# Autodesk Inventor assembly: (Unsaved)
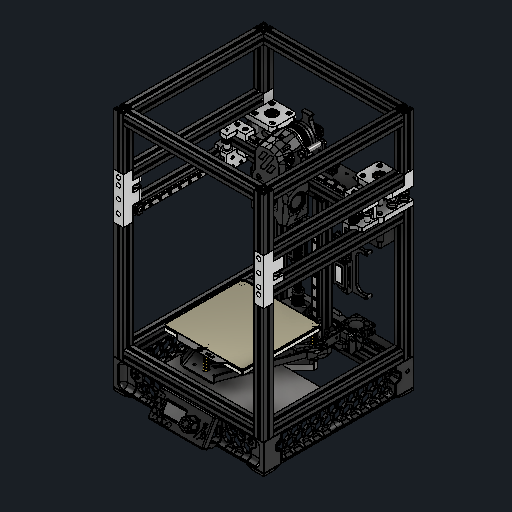
[picture p0: Inventor's stored thumbnail of the model, 512x512]
Saved by Autodesk Inventor 2026.2 (Build 302298000, 298)
## iProperties
Created: 2025-05-09
Part Number: (Unsaved)
Document SubType Name: Assembly
Designer: AdminForWorker
Title: Voron 0 v2
Author: AdminForWorker
## Documents named in this file (19)
- C:\Users\JoshuaEah\Documents\GitHub\Voron-0\CAD\Voron 0.iam
- C:\Users\JoshuaEah\Documents\GitHub\Voron-0\CAD\Frame\Frame.iam
- C:\Users\JoshuaEah\Documents\GitHub\Voron-0\CAD\Skirt\Skirts.iam
- C:\Users\JoshuaEah\Documents\GitHub\Voron-0\CAD\Hardware\Electronics\Electronics.iam
- C:\Users\JoshuaEah\Documents\GitHub\Voron-0\CAD\Extras\Filament Spool.iam
- C:\Users\JoshuaEah\Documents\GitHub\Voron-0\CAD\Z Axis\Bed Assembly.iam
- C:\Users\JoshuaEah\Documents\GitHub\Voron-0\CAD\Z Axis\Z Motor Assembly.iam
- C:\Users\JoshuaEah\Documents\GitHub\Voron-0\CAD\Z Axis\Z Extrusion Right.iam
- Z Extrusion Right.iam
- C:\Users\JoshuaEah\Documents\GitHub\Voron-0\CAD\Z Axis\Z Extrusion Left.iam
- C:\Users\JoshuaEah\Documents\GitHub\Voron-0\CAD\Hardware\Linear Rail\Parts\MGN7H Carriage.ipt
- C:\Users\JoshuaEah\Documents\GitHub\Voron-0\CAD\Belts\Belts.iam
- C:\Users\JoshuaEah\Documents\GitHub\Voron-0\CAD\X Axis\X Axis.iam
- C:\Users\JoshuaEah\Documents\GitHub\Voron-0\CAD\Toolhead\Mini Stealthburner.iam
- C:\Users\JoshuaEah\Documents\GitHub\Voron-0\CAD\Enclosure\Enclosure.iam
- C:\Users\JoshuaEah\Documents\GitHub\Voron-0\CAD\AB Drives\A_Drive.iam
- C:\Users\JoshuaEah\Documents\GitHub\Voron-0\CAD\AB Drives\B_Drive.iam
- C:\Users\JoshuaEah\Documents\GitHub\Voron-0\CAD\Idlers\A Idler Assembly (Alternate).iam
- C:\Users\JoshuaEah\Documents\GitHub\Voron-0\CAD\Idlers\B Idler Assembly (Alternate).iam
## Components (21 placed, 21 different names)
1. Frame:1 [sub-assembly] — Flush:3, Angle:1, Mate:4, Cylindrical:5, Insert:7, Insert:8, Mate:22, Mate:23, Angle:3, Cylindrical:13, Angle:4, Insert:17, Insert:18, Insert:19, Insert:20
2. Belts:1 [sub-assembly] — Mate:24
3. A_Drive:1 [sub-assembly] — Insert:7, Mate:23
4. B_Drive:1 [sub-assembly] — Insert:8, Mate:22
5. X Axis:1 [sub-assembly] — Insert:13, Insert:14, Cylindrical:12, Angle:2, Mate:24
6. MGN7H X Carriage:1 — Cylindrical:12, Insert:15, Insert:16, Angle:2
7. Mini Stealthburner:1 [sub-assembly] — Insert:15, Insert:16
8. MGN7H Y Left Carriage:1 — Cylindrical:5, Insert:13, Angle:3
9. MGN7H Y Right Carriage:1 — Insert:14, Cylindrical:13, Angle:4
10. Bed Assembly:1 [sub-assembly] — Mate:1, Insert:1, Insert:2, Insert:3, Insert:4
11. Z Motor Assembly:1 [sub-assembly] — Mate:1, Flush:3, Angle:1
12. Z Extrusion Right:1 [sub-assembly] — Cylindrical:15, Angle:6
13. Z Extrusion Left:1 [sub-assembly] — Mate:4, Cylindrical:14, Angle:5
14. MGN7H Z Left Carriage:1 — Insert:2, Insert:3, Cylindrical:14, Angle:5
15. MGN7H Z Right Carriage:1 — Insert:1, Insert:4, Cylindrical:15, Angle:6
16. Skirts:1 [sub-assembly]
17. Enclosure:1 [sub-assembly]
18. Electronics:1 [sub-assembly]
19. Filament Spool:1 [sub-assembly]
20. A Idler Assembly (Alternate):1 [sub-assembly] — Insert:17, Insert:18
21. B Idler Assembly (Alternate):1 [sub-assembly] — Insert:19, Insert:20
## Relationships (53: Mate 18, Insert 14, Flush 10, Angle 6, CylindricalJoint 5)
- Mate:1: Bed Assembly:1 ↔ Z Motor Assembly:1
- [Mate]: Frame:1 ↔ Z Extrusion Right:1
- [Mate]: Frame:1 ↔ Z Extrusion Left:1
- [Flush]: Frame:1 ↔ Z Extrusion Right:1
- [Flush]: Frame:1 ↔ Z Extrusion Left:1
- Insert:1: Bed Assembly:1 ↔ MGN7H Z Right Carriage:1
- Insert:2: Bed Assembly:1 ↔ MGN7H Z Left Carriage:1
- Insert:3: Bed Assembly:1 ↔ MGN7H Z Left Carriage:1
- Insert:4: Bed Assembly:1 ↔ MGN7H Z Right Carriage:1
- Flush:3: Frame:1 ↔ Z Motor Assembly:1
- Angle:1 (0 deg): Frame:1 ↔ Z Motor Assembly:1
- Mate:4 (58 mm): Frame:1 ↔ Z Extrusion Left:1
- [Flush]: Bed Assembly:1 ↔ Z Extrusion Right:1
- Cylindrical:5: Frame:1 ↔ MGN7H Y Left Carriage:1
- [Mate]: Frame:1 ↔ Enclosure:1
- [Flush]: Frame:1 ↔ Enclosure:1
- [Flush]: Frame:1 ↔ Enclosure:1
- [Mate]: Frame:1 ↔ Enclosure:1
- [Flush]: Frame:1 ↔ Enclosure:1
- [Flush]: Frame:1 ↔ Enclosure:1
- [Mate]: Frame:1 ↔ Enclosure:1
- [Flush]: Frame:1 ↔ Enclosure:1
- [Flush]: Frame:1 ↔ Enclosure:1
- [Mate] (0.5 mm): Frame:1 ↔ Enclosure:1
- [Mate] (1 mm): Frame:1 ↔ Enclosure:1
- [Mate] (0.5 mm): Frame:1 ↔ Enclosure:1
- [Mate] (0.5 mm): Frame:1 ↔ Enclosure:1
- [Mate] (0.5 mm): Frame:1 ↔ Enclosure:1
- [Mate] (0.5 mm): Frame:1 ↔ Enclosure:1
- [Mate] (0.5 mm): Frame:1 ↔ Enclosure:1
- [Mate] (0.5 mm): Frame:1 ↔ Enclosure:1
- Insert:7: Frame:1 ↔ A_Drive:1
- Insert:8: Frame:1 ↔ B_Drive:1
- Mate:22: Frame:1 ↔ B_Drive:1
- Mate:23: Frame:1 ↔ A_Drive:1
- Insert:13: X Axis:1 ↔ MGN7H Y Left Carriage:1
- Insert:14: X Axis:1 ↔ MGN7H Y Right Carriage:1
- Cylindrical:12: X Axis:1 ↔ MGN7H X Carriage:1
- Insert:15: MGN7H X Carriage:1 ↔ Mini Stealthburner:1
- Insert:16: MGN7H X Carriage:1 ↔ Mini Stealthburner:1
- Angle:2 (0 deg): X Axis:1 ↔ MGN7H X Carriage:1
- Angle:3 (0 deg): Frame:1 ↔ MGN7H Y Left Carriage:1
- Cylindrical:13: Frame:1 ↔ MGN7H Y Right Carriage:1
- Angle:4 (0 deg): Frame:1 ↔ MGN7H Y Right Carriage:1
- Cylindrical:14: Z Extrusion Left:1 ↔ MGN7H Z Left Carriage:1
- Angle:5 (0 deg): Z Extrusion Left:1 ↔ MGN7H Z Left Carriage:1
- Cylindrical:15: Z Extrusion Right:1 ↔ MGN7H Z Right Carriage:1
- Angle:6 (0 deg): Z Extrusion Right:1 ↔ MGN7H Z Right Carriage:1
- Insert:17: Frame:1 ↔ A Idler Assembly (Alternate):1
- Insert:18: Frame:1 ↔ A Idler Assembly (Alternate):1
- Insert:19: Frame:1 ↔ B Idler Assembly (Alternate):1
- Insert:20: Frame:1 ↔ B Idler Assembly (Alternate):1
- Mate:24: Belts:1 ↔ X Axis:1
